# Autodesk Inventor assembly: Shooter Curve Assembly
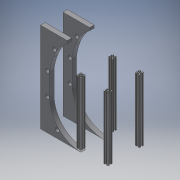
[picture p0: Inventor's stored thumbnail of the model, 180x180]
Saved by Autodesk Inventor 2018 (Build 220112000, 112)
## iProperties
Created: 2020-02-01
Part Number: Shooter Curve Assembly
Document SubType Name: Assembly
Designer: Weeb No1
Author: Weeb No1
## Documents named in this file (3)
- C:\Users\Weeb No1\Documents\GitHub\2020CAD\Gabriel Inventor Files (Shooter, Drivebase)\Shooter Curve Assembly\Main Assembly File\Shooter Curve Assembly.iam
- C:\Users\Weeb No1\Documents\GitHub\2020CAD\Gabriel Inventor Files (Shooter, Drivebase)\Shooter Curve Assembly\Part Files\Part3.ipt
- C:\Users\Weeb No1\Documents\GitHub\2020CAD\Gabriel Inventor Files (Shooter, Drivebase)\Shooter Curve Assembly\Part Files\8020 1010 x 14.ipt
## Components (6 placed, 2 different names)
1. Part3:1 — Flush:1, Mate:1, Mate:2, Flush:2, Flush:3
2. 8020 1010 x 14:1 — Flush:1, Mate:1, Mate:4, Flush:5, Flush:6, Flush:9
3. 8020 1010 x 14:2 — Flush:4, Mate:3, Mate:5, Flush:7, Flush:8, Flush:9
4. Part3:2 — Mate:2, Flush:2, Flush:3, Flush:4, Mate:3
5. 8020 1010 x 14:3 — Mate:4, Flush:5, Flush:6, Flush:10
6. 8020 1010 x 14:4 — Mate:5, Flush:7, Flush:8, Flush:10
## Relationships (15: Flush 10, Mate 5)
- Flush:1 (228.6 mm): Part3:1 ↔ 8020 1010 x 14:1
- Mate:1: Part3:1 ↔ 8020 1010 x 14:1
- Mate:2 (101.6 mm): Part3:1 ↔ Part3:2
- Flush:2: Part3:1 ↔ Part3:2
- Flush:3: Part3:1 ↔ Part3:2
- Flush:4 (228.6 mm): 8020 1010 x 14:2 ↔ Part3:2
- Mate:3: 8020 1010 x 14:2 ↔ Part3:2
- Mate:4 (127 mm): 8020 1010 x 14:1 ↔ 8020 1010 x 14:3
- Flush:5: 8020 1010 x 14:1 ↔ 8020 1010 x 14:3
- Flush:6: 8020 1010 x 14:1 ↔ 8020 1010 x 14:3
- Mate:5 (127 mm): 8020 1010 x 14:2 ↔ 8020 1010 x 14:4
- Flush:7: 8020 1010 x 14:2 ↔ 8020 1010 x 14:4
- Flush:8: 8020 1010 x 14:2 ↔ 8020 1010 x 14:4
- Flush:9: 8020 1010 x 14:1 ↔ 8020 1010 x 14:2
- Flush:10: 8020 1010 x 14:3 ↔ 8020 1010 x 14:4
